# Autodesk Inventor assembly: БН
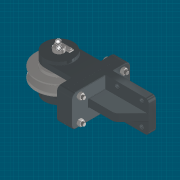
[picture p0: Inventor's stored thumbnail of the model, 180x180]
Saved by Autodesk Inventor 2021.2 (Build 252289000, 289)
## iProperties
Created: 2022-05-01
Part Number: БН
Document SubType Name: Assembly
Designer: DuctopwH
Author: DuctopwH
## Documents named in this file (11)
- F:\Projects\cadblueprints\004-БН\004-BN.iam
- F:\Projects\cadblueprints\004-БН\parts\004.00.01-rolik.ipt
- F:\Projects\cadblueprints\004-БН\parts\004.00.04-vtulka.ipt
- F:\Projects\cadblueprints\004-БН\parts\004.00.02-vilka.ipt
- F:\Projects\cadblueprints\004-БН\parts\004.00.03-kronshtein.ipt
- C:\Users\DuctopwH\Documents\Inventor\Content Center Files\R2021\en-US\Screw GOST 1477-93\Screw A.M8-6gx16 GOST 1477-93.ipt
- F:\Projects\cadblueprints\004-БН\parts\004.00.06-os.ipt
- F:\Projects\cadblueprints\004-БН\parts\004.00.05-planka.ipt
- C:\Users\DuctopwH\Documents\Inventor\Content Center Files\R2021\en-US\Bolt A GOST 7811-70\Bolt A M6-6g×30 GOST 7811-70.ipt
- C:\Users\DuctopwH\Documents\Inventor\Content Center Files\R2021\en-US\GOST 5915-70\Nut M12-6H GOST 5915-70(1).ipt
- C:\Users\DuctopwH\Documents\Inventor\Content Center Files\R2021\en-US\GOST 7805-70\Bolt M12-6gx70 GOST 7805-70.ipt
## Components (17 placed, 10 different names)
1. 004.00.01-rolik:1 — Mate:1, Mate:2, Flush:1, Mate:33, Flush:2, Flush:35
2. 004.00.04-vtulka:1 — Mate:1, Mate:2, Mate:13, Mate:32
3. 004.00.03-kronshtein:1 — Mate:10, Mate:11, Mate:12, Insert:1, Insert:2, Insert:3, Insert:4
4. Screw GOST 1477-93 M8x16-A:1 — Mate:32, Mate:33, Flush:2
5. 004.00.02-vilka:1 — Mate:10, Mate:11, Mate:12, Mate:13, Mate:14, Mate:15, Mate:16, Mate:17, Mate:18, Mate:19, Mate:20, Mate:21, Mate:22, Mate:23, Mate:24, Mate:25, Mate:26
6. 004.00.06-os:1 — Mate:14, Mate:15, Mate:27
7. 004.00.05-planka:1 — Mate:16, Mate:17, Mate:18, Mate:27, Mate:28, Mate:29, Mate:30, Mate:31
8. Bolt GOST 7805-70 M12-6gx70:1 — Mate:21, Mate:26
9. Bolt GOST 7805-70 M12-6gx70:2 — Mate:19, Mate:20
10. Bolt GOST 7805-70 M12-6gx70:3 — Mate:22, Mate:25
11. Bolt GOST 7805-70 M12-6gx70:4 — Mate:23, Mate:24
12. Bolt A GOST 7811-70 M6-6g×30:2 — Mate:28, Mate:29
13. Nut GOST 5915-70 M12:1 — Insert:1
14. Nut GOST 5915-70 M12:2 — Insert:2
15. Nut GOST 5915-70 M12:3 — Insert:3
16. Nut GOST 5915-70 M12:4 — Insert:4
17. Bolt A GOST 7811-70 M6-6g×30:3 — Mate:30, Mate:31
## Relationships (33: Mate 26, Insert 4, Flush 3)
- Mate:1: 004.00.01-rolik:1 ↔ 004.00.04-vtulka:1
- Mate:2: 004.00.01-rolik:1 ↔ 004.00.04-vtulka:1
- Mate:10: 004.00.03-kronshtein:1 ↔ 004.00.02-vilka:1
- Mate:11: 004.00.03-kronshtein:1 ↔ 004.00.02-vilka:1
- Mate:12: 004.00.03-kronshtein:1 ↔ 004.00.02-vilka:1
- Flush:1: 004.00.01-rolik:1
- Mate:13: 004.00.04-vtulka:1 ↔ 004.00.02-vilka:1
- Mate:14: 004.00.02-vilka:1 ↔ 004.00.06-os:1
- Mate:15: 004.00.02-vilka:1 ↔ 004.00.06-os:1
- Mate:16: 004.00.02-vilka:1 ↔ 004.00.05-planka:1
- Mate:17: 004.00.02-vilka:1 ↔ 004.00.05-planka:1
- Mate:18: 004.00.02-vilka:1 ↔ 004.00.05-planka:1
- Mate:19: 004.00.02-vilka:1 ↔ Bolt GOST 7805-70 M12-6gx70:2
- Mate:20: 004.00.02-vilka:1 ↔ Bolt GOST 7805-70 M12-6gx70:2
- Mate:21: 004.00.02-vilka:1 ↔ Bolt GOST 7805-70 M12-6gx70:1
- Mate:22: 004.00.02-vilka:1 ↔ Bolt GOST 7805-70 M12-6gx70:3
- Mate:23: 004.00.02-vilka:1 ↔ Bolt GOST 7805-70 M12-6gx70:4
- Mate:24: 004.00.02-vilka:1 ↔ Bolt GOST 7805-70 M12-6gx70:4
- Mate:25: 004.00.02-vilka:1 ↔ Bolt GOST 7805-70 M12-6gx70:3
- Mate:26: 004.00.02-vilka:1 ↔ Bolt GOST 7805-70 M12-6gx70:1
- Mate:27: 004.00.06-os:1 ↔ 004.00.05-planka:1
- Mate:28: 004.00.05-planka:1 ↔ Bolt A GOST 7811-70 M6-6g×30:2
- Mate:29: 004.00.05-planka:1 ↔ Bolt A GOST 7811-70 M6-6g×30:2
- Insert:1: 004.00.03-kronshtein:1 ↔ Nut GOST 5915-70 M12:1
- Insert:2: 004.00.03-kronshtein:1 ↔ Nut GOST 5915-70 M12:2
- Insert:3: 004.00.03-kronshtein:1 ↔ Nut GOST 5915-70 M12:3
- Insert:4: 004.00.03-kronshtein:1 ↔ Nut GOST 5915-70 M12:4
- Mate:30: 004.00.05-planka:1 ↔ Bolt A GOST 7811-70 M6-6g×30:3
- Mate:31: 004.00.05-planka:1 ↔ Bolt A GOST 7811-70 M6-6g×30:3
- Mate:32: 004.00.04-vtulka:1 ↔ Screw GOST 1477-93 M8x16-A:1
- Mate:33: 004.00.01-rolik:1 ↔ Screw GOST 1477-93 M8x16-A:1
- Flush:2: 004.00.01-rolik:1 ↔ Screw GOST 1477-93 M8x16-A:1
- Flush:35: 004.00.01-rolik:1
